# Autodesk Inventor assembly: Motor mount assembly
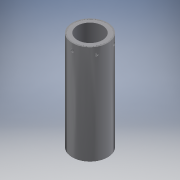
[picture p0: Inventor's stored thumbnail of the model, 180x180]
Saved by Autodesk Inventor 2019 (Build 230136000, 136)
## iProperties
Created: 2023-01-20
Part Number: Motor mount assembly
Document SubType Name: Assembly
Designer: user
Author: user
## Documents named in this file (3)
- C:\Users\user\Documents\Water Desalinator\Motor mount assembly.iam
- C:\Users\user\Documents\Water Desalinator\Motor mount.ipt
- C:\Users\user\Documents\Water Desalinator\Tail tube.ipt
## Components (2 placed, 2 different names)
1. Motor mount:1 — Cylindrical:1, Mate:1
2. Tail tube:1 — Cylindrical:1, Mate:1
## Relationships (3: CylindricalJoint 1, Mate 1, Symmetry 1)
- Cylindrical:1: Motor mount:1 ↔ Tail tube:1
- Mate:1: Motor mount:1 ↔ Tail tube:1
- Symmetry:1
